# Autodesk Inventor assembly: ASY GnG station
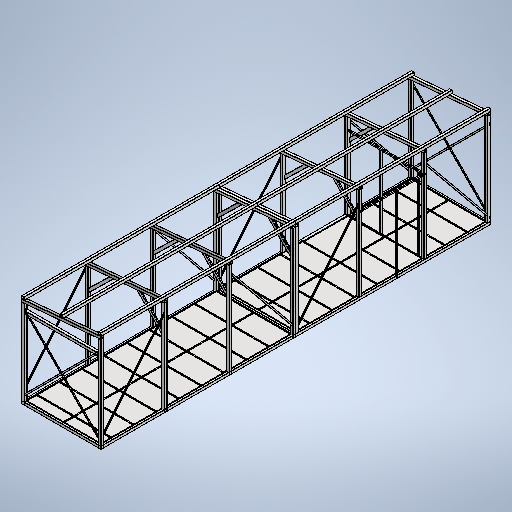
[picture p0: Inventor's stored thumbnail of the model, 512x512]
Saved by Autodesk Inventor 2025.3 (Build 293356000, 356)
## iProperties
Created: 2025-09-20
Part Number: ASY GnG station
Document SubType Name: Assembly
Designer: admin
Mass: 1.79457e+07 g
Surface Area: 4.32168e+06 cm^2
Volume: 1.64264e+07 cm^3
Density: 1.0925 g/cm^3
Author: admin
## Documents named in this file (9)
- C:\Users\admin\Yandex.Disk\home pc\Inventor\GnG_Gantul_hill\ASY GnG station.iam
- C:\Users\admin\Yandex.Disk\home pc\Inventor\GnG_Gantul_hill\GNG НаOCl pan.ipt
- C:\Users\admin\Yandex.Disk\home pc\Inventor\GnG_Gantul_hill\GNG НаOCl tank 2.ipt
- C:\Users\admin\Yandex.Disk\home pc\Inventor\GnG_Gantul_hill\GNG НаOCl tank 2_MIR.ipt
- C:\Users\admin\Yandex.Disk\home pc\Inventor\GnG_Gantul_hill\ASY GnG frame 2.iam
- C:\Users\admin\Yandex.Disk\home pc\Inventor\GnG_Gantul_hill\ASY GnG frame 1.1.iam
- C:\Users\admin\Yandex.Disk\home pc\Inventor\GnG_Gantul_hill\GnG- -Sandwich wall.ipt
- C:\Users\admin\Yandex.Disk\home pc\Inventor\GnG_Gantul_hill\GnG- -Sandwich roof.ipt
- C:\Users\admin\Yandex.Disk\home pc\Inventor\GnG_Gantul_hill\GnG- -Sandwich wall low.ipt
## Components (37 placed, 8 different names)
1. GNG НаOCl pan:1 — Mate:6, Flush:2, Tangent:1, Mate:9, Rigid:1, Mate:10, Mate:11
2. GNG НаOCl pan:2 — Flush:2, Rigid:1, Flush:3
3. GNG НаOCl tank 2:1 — Mate:6, Tangent:1, Mate:9, Rigid:2
4. GNG НаOCl tank 2_MIR:1 — Rigid:2
5. ASY GnG frame 2:1 [sub-assembly] — Rigid:3, Mate:12, Flush:4, Mate:16, Flush:9
6. ASY GnG frame 1.1:1 [sub-assembly] — Rigid:3, Mate:10, Mate:11, Flush:3, Mate:14, Flush:5, Mate:15, Flush:6, Flush:8
7. GnG- -Sandwich wall:11 — Mate:16, Flush:9, Rigid:4
8. GnG- -Sandwich wall:12 — Rigid:4
9. GnG- -Sandwich roof:1 — Mate:12, Flush:4
10. GnG- -Sandwich roof:2
11. GnG- -Sandwich roof:3
12. GnG- -Sandwich roof:4
13. GnG- -Sandwich roof:5
14. GnG- -Sandwich roof:6
15. GnG- -Sandwich roof:7
16. GnG- -Sandwich roof:8
17. GnG- -Sandwich roof:9
18. GnG- -Sandwich roof:10
19. GnG- -Sandwich roof:11
20. GnG- -Sandwich wall low:1 — Mate:15, Flush:6, Flush:7
21. GnG- -Sandwich wall low:2
22. GnG- -Sandwich wall low:3
23. GnG- -Sandwich wall low:4
24. GnG- -Sandwich wall low:5
25. GnG- -Sandwich wall low:6
26. GnG- -Sandwich wall low:7
27. GnG- -Sandwich wall low:8
28. GnG- -Sandwich wall low:9
29. GnG- -Sandwich wall:1 — Mate:14, Flush:5, Flush:7, Flush:8
30. GnG- -Sandwich wall:13
31. GnG- -Sandwich wall:14
32. GnG- -Sandwich wall:15
33. GnG- -Sandwich wall:16
34. GnG- -Sandwich wall:17
35. GnG- -Sandwich wall:18
36. GnG- -Sandwich wall:19
37. GnG- -Sandwich wall:20
## Component patterns: (11 elements, first: GnG- -Sandwich roof:1), (9 elements, first: GnG- -Sandwich wall low:1), (9 elements, first: GnG- -Sandwich wall:1)
## Relationships (21: Mate 8, Flush 8, WeldJoint 4, Tangent 1)
- Mate:6 (40 mm): GNG НаOCl pan:1 ↔ GNG НаOCl tank 2:1
- Flush:2: GNG НаOCl pan:1 ↔ GNG НаOCl pan:2
- Tangent:1 (50 mm): GNG НаOCl pan:1 ↔ GNG НаOCl tank 2:1
- Mate:9: GNG НаOCl pan:1 ↔ GNG НаOCl tank 2:1
- Rigid:1 [WeldJoint] (400 mm): GNG НаOCl pan:1 ↔ GNG НаOCl pan:2
- Rigid:2 [WeldJoint] (600 mm): GNG НаOCl tank 2:1 ↔ GNG НаOCl tank 2_MIR:1
- Rigid:3 [WeldJoint]: ASY GnG frame 2:1 ↔ ASY GnG frame 1.1:1
- Mate:10: GNG НаOCl pan:1 ↔ ASY GnG frame 1.1:1
- Mate:11: GNG НаOCl pan:1 ↔ ASY GnG frame 1.1:1
- Flush:3 (400 mm): GNG НаOCl pan:2 ↔ ASY GnG frame 1.1:1
- Mate:12: ASY GnG frame 2:1 ↔ GnG- -Sandwich roof:1
- Flush:4 (-100 mm): ASY GnG frame 2:1 ↔ GnG- -Sandwich roof:1
- Mate:14: ASY GnG frame 1.1:1 ↔ GnG- -Sandwich wall:1
- Flush:5: ASY GnG frame 1.1:1 ↔ GnG- -Sandwich wall:1
- Mate:15: ASY GnG frame 1.1:1 ↔ GnG- -Sandwich wall low:1
- Flush:6: ASY GnG frame 1.1:1 ↔ GnG- -Sandwich wall low:1
- Flush:7: GnG- -Sandwich wall low:1 ↔ GnG- -Sandwich wall:1
- Flush:8: ASY GnG frame 1.1:1 ↔ GnG- -Sandwich wall:1
- Mate:16: ASY GnG frame 2:1 ↔ GnG- -Sandwich wall:11
- Flush:9: ASY GnG frame 2:1 ↔ GnG- -Sandwich wall:11
- Rigid:4 [WeldJoint]: GnG- -Sandwich wall:11 ↔ GnG- -Sandwich wall:12
